# Autodesk Inventor assembly: encoder
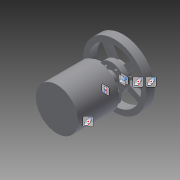
[picture p0: Inventor's stored thumbnail of the model, 180x180]
Saved by Autodesk Inventor 2015 (Build 190159000, 159)
## iProperties
Created: 2015-07-19
Part Number: encoder
Document SubType Name: Assembly
Designer: astralien3000
Author: astralien3000
## Documents named in this file (4)
- C:\Users\astralien3000\Desktop\ceres\meca\v2016\encoder.iam
- C:\Users\astralien3000\Desktop\ceres\meca\lib\wheel\pololu_wheel_60x8.ipt
- C:\Users\astralien3000\Desktop\ceres\meca\lib\struct\hub_6mm_M3.ipt
- C:\Users\astralien3000\Desktop\ceres\meca\lib\sensor\encoder_E6B2.ipt
## Components (3 placed, 3 different names)
1. pololu_wheel_60x8:1 — Placage:2, Placage:3, Placage:5
2. hub_6mm_M3:1 — Placage:2, Placage:3, Placage:4
3. encoder_E6B2:1 — Placage:1, Affleurement:1, Placage:4, Placage:5
## Relationships (6: Mate 5, Flush 1)
- Placage:1 [Mate]: encoder_E6B2:1
- Affleurement:1 [Flush]: encoder_E6B2:1
- Placage:2 [Mate]: pololu_wheel_60x8:1 ↔ hub_6mm_M3:1
- Placage:3 [Mate]: pololu_wheel_60x8:1 ↔ hub_6mm_M3:1
- Placage:4 [Mate]: hub_6mm_M3:1 ↔ encoder_E6B2:1
- Placage:5 [Mate] (10.8 mm): pololu_wheel_60x8:1 ↔ encoder_E6B2:1
